# Autodesk Inventor assembly: IDC10Combine2
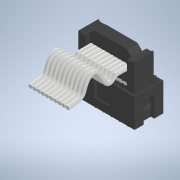
[picture p0: Inventor's stored thumbnail of the model, 180x180]
Saved by Autodesk Inventor 2021 (Build 250183000, 183)
## iProperties
Created: 2023-08-07
Part Number: IDC10Combine2
Document SubType Name: Assembly
Designer: michal
Author: michal
## Documents named in this file (4)
- C:\Users\micha\OneDrive\Dokumenty\GitHub\escape_room_hw_v2\Enclosure\Commercial\IDC10Combine2.iam
- C:\Users\micha\Downloads\61201023021.iam
- C:\Users\micha\Downloads\ribbonAss.iam
- C:\Users\micha\OneDrive\Dokumenty\GitHub\escape_room_hw_v2\Enclosure\Commercial\139366252-9-61201021621\61201021621.iam
## Components (3 placed, 3 different names)
1. 61201023021:1 [sub-assembly] — Mate:1, Mate:2, Mate:3, Mate:4, Flush:1, Mate:5
2. ribbonAss:1 [sub-assembly] — Mate:4, Flush:1, Mate:5
3. 61201021621:1 [sub-assembly] — Mate:1, Mate:2, Mate:3
## Relationships (6: Mate 5, Flush 1)
- Mate:1: 61201023021:1 ↔ 61201021621:1
- Mate:2: 61201023021:1 ↔ 61201021621:1
- Mate:3: 61201023021:1 ↔ 61201021621:1
- Mate:4: 61201023021:1 ↔ ribbonAss:1
- Flush:1: 61201023021:1 ↔ ribbonAss:1
- Mate:5: 61201023021:1 ↔ ribbonAss:1
